# Autodesk Inventor assembly: assembly
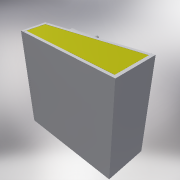
[picture p0: Inventor's stored thumbnail of the model, 180x180]
Saved by Autodesk Inventor 2017 (Build 210142000, 142)
## iProperties
Created: 2017-03-04
Part Number: assembly
Document SubType Name: Assembly
Designer: dpgai
Author: dpgai
## Documents named in this file (14)
- C:\Users\dpgai\Documents\Inventor\MIDI_proj\assembly.iam
- C:\Users\dpgai\Documents\Inventor\MIDI_proj\bottom.ipt
- C:\Users\dpgai\Documents\Inventor\MIDI_proj\sides.ipt
- C:\Users\dpgai\Documents\Inventor\MIDI_proj\top.ipt
- C:\Users\dpgai\Documents\Inventor\MIDI_proj\back.ipt
- C:\Users\dpgai\Documents\Inventor\MIDI_proj\front.ipt
- C:\Users\dpgai\Documents\Inventor\MIDI_proj\Potentiometer knob.ipt
- C:\Users\dpgai\Documents\Inventor\MIDI_proj\B10K potentiometer 10K.ipt
- C:\Users\dpgai\Documents\Inventor\MIDI_proj\LTL2T3TGK6.iam
- C:\Users\dpgai\Documents\Inventor\MIDI_proj\LED holder.ipt
- C:\Users\dpgai\Documents\Inventor\MIDI_proj\ISO 7380-1 M3x16mm.ipt
- C:\Users\dpgai\Documents\Inventor\MIDI_proj\10K Linear Pot - 770-3131.ipt
- C:\Users\dpgai\Documents\Inventor\MIDI_proj\Adafruit Trellis 3mm.ipt
- C:\Users\dpgai\Documents\Inventor\MIDI_proj\pot slider.ipt
## Components (27 placed, 13 different names)
1. bottom:1 — Mate:2, Flush:2, Flush:3, Flush:4, Mate:3, Flush:5, Flush:9, Flush:10
2. sides:1 — Flush:4, Mate:3, Flush:5
3. top:1 — Mate:4, Flush:12, Flush:13, Flush:14, Flush:15, Mate:5, Insert:1, Insert:3, Insert:5, Mate:6, Mate:7, Mate:8, Mate:9, Mate:10, Mate:11, Mate:12
4. sides:2 — Mate:2, Flush:2, Flush:3, Flush:8, Flush:11, Flush:12, Mate:5
5. back:1 — Flush:10, Flush:11, Flush:13, Flush:15
6. front:1 — Flush:8, Flush:9, Mate:4, Flush:14
7. Adafruit Trellis 3mm:1 — Mate:9, Mate:10, Mate:11
8. B10K potentiometer 10K:1 — Insert:1, Insert:2
9. B10K potentiometer 10K:2
10. B10K potentiometer 10K:3
11. B10K potentiometer 10K:4
12. Potentiometer knob:1 — Insert:2
13. Potentiometer knob:2
14. Potentiometer knob:3
15. Potentiometer knob:4
16. LTL2T3TGK6:1 [sub-assembly] — Insert:4
17. LED holder:1 — Insert:3, Insert:4
18. LTL2T3TGK6:2 [sub-assembly]
19. LED holder:2
20. ISO 7380-1 M3x16mm:1 — Insert:5
21. ISO 7380-1 M3x16mm:2
22. ISO 7380-1 M3x16mm:3
23. ISO 7380-1 M3x16mm:4
24. 10K Linear Pot - 770-3131:1 — Mate:6, Mate:7, Mate:8, Mate:13
25. 10K Linear Pot - 770-3131:2
26. pot slider:1 — Mate:12, Mate:13
27. pot slider:2
## Component patterns: (4 elements, first: B10K potentiometer 10K:1), (4 elements, first: Potentiometer knob:1), (2 elements, first: LTL2T3TGK6:1 + LED holder:1), (4 elements, first: ISO 7380-1 M3x16mm:1), (2 elements, first: 10K Linear Pot - 770-3131:1), (2 elements, first: pot slider:1)
## Relationships (29: Mate 12, Flush 12, Insert 5)
- Mate:2: bottom:1 ↔ sides:2
- Flush:2: bottom:1 ↔ sides:2
- Flush:3: bottom:1 ↔ sides:2
- Flush:4: bottom:1 ↔ sides:1
- Mate:3: bottom:1 ↔ sides:1
- Flush:5: bottom:1 ↔ sides:1
- Flush:8: sides:2 ↔ front:1
- Flush:9: bottom:1 ↔ front:1
- Flush:10: bottom:1 ↔ back:1
- Flush:11: sides:2 ↔ back:1
- Mate:4: top:1 ↔ front:1
- Flush:12: top:1 ↔ sides:2
- Flush:13: top:1 ↔ back:1
- Flush:14: top:1 ↔ front:1
- Flush:15: top:1 ↔ back:1
- Mate:5: top:1 ↔ sides:2
- Insert:1: top:1 ↔ B10K potentiometer 10K:1
- Insert:2: B10K potentiometer 10K:1 ↔ Potentiometer knob:1
- Insert:3: top:1 ↔ LED holder:1
- Insert:4: LTL2T3TGK6:1 ↔ LED holder:1
- Insert:5: top:1 ↔ ISO 7380-1 M3x16mm:1
- Mate:6: top:1 ↔ 10K Linear Pot - 770-3131:1
- Mate:7: top:1 ↔ 10K Linear Pot - 770-3131:1
- Mate:8: top:1 ↔ 10K Linear Pot - 770-3131:1
- Mate:9: top:1 ↔ Adafruit Trellis 3mm:1
- Mate:10: top:1 ↔ Adafruit Trellis 3mm:1
- Mate:11: top:1 ↔ Adafruit Trellis 3mm:1
- Mate:12: top:1 ↔ pot slider:1
- Mate:13: 10K Linear Pot - 770-3131:1 ↔ pot slider:1
